# Autodesk Inventor assembly: Standard Wheel Assembly V2
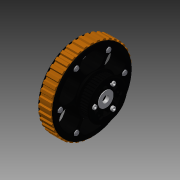
[picture p0: Inventor's stored thumbnail of the model, 180x180]
Saved by Autodesk Inventor 2013 (Build 170138000, 138)
## iProperties
Created: 2013-01-17
Part Number: Standard Wheel Assembly V2
Document SubType Name: Assembly
Designer: Moses
Mass: 472.813 g
Surface Area: 1601.3 cm^2
Volume: 372.815 cm^3
Density: 1.26822 g/cm^3
Author: Moses
## Documents named in this file (6)
- C:\Users\Moses\Documents\GitHub\frc2013CAD\Drivetrain\Standard Wheel Assembly V2.iam
- C:\Users\Moses\Documents\GitHub\frc2013CAD\Drivetrain\6Plaction-asm\6Plaction-asm.iam
- C:\Users\Moses\Documents\GitHub\frc2013CAD\Drivetrain\DBK_42ToothPulley (am-2234)\DBK_42ToothPulley V2.iam
- C:\Users\Moses\Documents\GitHub\frc2013CAD\Drivetrain\DBK_42ToothPulley (am-2234)\Belt Pulley Spacer.ipt
- C:\Users\Moses\Documents\GitHub\frc2013CAD\Drivetrain\Bearings\r8 bearing.ipt
- C:\Users\Moses\Documents\GitHub\frc2013CAD\Drivetrain\91251A255 10-24 Screw\91251A255.ipt
## Components (13 placed, 5 different names)
1. 6Plaction-asm:1 [sub-assembly] — Mate:1, Mate:2, Mate:3, Insert:8
2. DBK_42ToothPulley V2:2 [sub-assembly] — Insert:1, Insert:2, Insert:3, Insert:4, Insert:5, Insert:6, Mate:2, Mate:3, Insert:7, Insert:9, Insert:10, Insert:11
3. Belt Pulley Spacer:1 — Insert:1
4. Belt Pulley Spacer:2 — Insert:2, Mate:1
5. Belt Pulley Spacer:3 — Insert:3
6. Belt Pulley Spacer:4 — Insert:4
7. Belt Pulley Spacer:5 — Insert:5
8. Belt Pulley Spacer:6 — Insert:6
9. r8 bearing:1 — Insert:7
10. r8 bearing:2 — Insert:8
11. 91251A255:1 — Insert:9
12. 91251A255:2 — Insert:10
13. 91251A255:3 — Insert:11
## Relationships (14: Insert 11, Mate 3)
- Insert:1: DBK_42ToothPulley V2:2 ↔ Belt Pulley Spacer:1
- Insert:2: DBK_42ToothPulley V2:2 ↔ Belt Pulley Spacer:2
- Insert:3: DBK_42ToothPulley V2:2 ↔ Belt Pulley Spacer:3
- Insert:4: DBK_42ToothPulley V2:2 ↔ Belt Pulley Spacer:4
- Insert:5: DBK_42ToothPulley V2:2 ↔ Belt Pulley Spacer:5
- Insert:6: DBK_42ToothPulley V2:2 ↔ Belt Pulley Spacer:6
- Mate:1: 6Plaction-asm:1 ↔ Belt Pulley Spacer:2
- Mate:2: 6Plaction-asm:1 ↔ DBK_42ToothPulley V2:2
- Mate:3: 6Plaction-asm:1 ↔ DBK_42ToothPulley V2:2
- Insert:7: DBK_42ToothPulley V2:2 ↔ r8 bearing:1
- Insert:8: 6Plaction-asm:1 ↔ r8 bearing:2
- Insert:9: DBK_42ToothPulley V2:2 ↔ 91251A255:1
- Insert:10: DBK_42ToothPulley V2:2 ↔ 91251A255:2
- Insert:11: DBK_42ToothPulley V2:2 ↔ 91251A255:3
